# Autodesk Inventor assembly: GANTRY
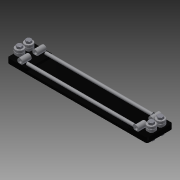
[picture p0: Inventor's stored thumbnail of the model, 180x180]
Saved by Autodesk Inventor 2013 (Build 170138000, 138)
## iProperties
Created: 2014-03-03
Part Number: GANTRY
Document SubType Name: Assembly
Designer: employee
Author: employee
## Documents named in this file (3)
- C:\Users\employee\Desktop\CoreXZ\GANTRY.iam
- C:\Users\employee\Desktop\CoreXZ\HALF GANTRY ASSEMBLY.iam
- C:\Users\employee\Desktop\CoreXZ\GANTRY CROSS PLATE.ipt
## Components (3 placed, 2 different names)
1. HALF GANTRY ASSEMBLY:1 [sub-assembly] — Insert:1, Insert:2, Flush:1
2. HALF GANTRY ASSEMBLY:2 [sub-assembly] — Insert:1, Insert:2
3. GANTRY CROSS PLATE:1 — Flush:1
## Relationships (3: Insert 2, Flush 1)
- Insert:1: HALF GANTRY ASSEMBLY:1 ↔ HALF GANTRY ASSEMBLY:2
- Insert:2: HALF GANTRY ASSEMBLY:1 ↔ HALF GANTRY ASSEMBLY:2
- Flush:1: HALF GANTRY ASSEMBLY:1 ↔ GANTRY CROSS PLATE:1
